# Autodesk Inventor assembly: ModularBrainsv2
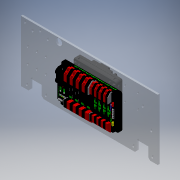
[picture p0: Inventor's stored thumbnail of the model, 180x180]
Saved by Autodesk Inventor 2018 (Build 220112000, 112)
## iProperties
Created: 2017-09-12
Part Number: ModularBrainsv2
Document SubType Name: Assembly
Designer: Srinity
Author: Srinity
## Documents named in this file (4)
- C:\Users\Srinity\Documents\DIY Projects\ModularFRCPlatform\ModularBrainsv2.iam
- C:\Users\Srinity\Documents\DIY Projects\ModularFRCPlatform\LexanPlate.ipt
- C:\Users\Srinity\Documents\DIY Projects\ModularFRCPlatform\14-806880.ipt
- C:\Users\Srinity\Documents\DIY Projects\ModularFRCPlatform\155213D-01L.ipt
## Components (3 placed, 3 different names)
1. LexanPlate:1 — Mate:1, Mate:2, Mate:3, Mate:4, Mate:5, Mate:6
2. 14-806880:1 — Mate:1, Mate:2, Mate:3
3. 155213D-01L:1 — Mate:4, Mate:5, Mate:6
## Relationships (6: Mate 6)
- Mate:1: LexanPlate:1 ↔ 14-806880:1
- Mate:2: LexanPlate:1 ↔ 14-806880:1
- Mate:3: LexanPlate:1 ↔ 14-806880:1
- Mate:4: LexanPlate:1 ↔ 155213D-01L:1
- Mate:5: LexanPlate:1 ↔ 155213D-01L:1
- Mate:6: LexanPlate:1 ↔ 155213D-01L:1
